# Autodesk Inventor assembly: assy-scara_new_components
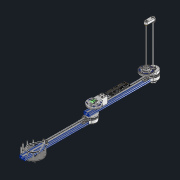
[picture p0: Inventor's stored thumbnail of the model, 180x180]
Saved by Autodesk Inventor 2022 (Build 260153000, 153)
## iProperties
Created: 2021-10-09
Part Number: assy-scara_new_components
Document SubType Name: Assembly
Designer: Yuta Kage
Mass: 10035.1 g
Surface Area: 20178.9 cm^2
Volume: 3427.41 cm^3
Density: 2.92791 g/cm^3
Author: Yuta Kage
## Documents named in this file (5)
- C:\Users\yuta0\Desktop\assy-scara\assy-scara_new_components.iam
- C:\Users\yuta0\Desktop\assy-scara\s-assy-linear_joint.iam
- C:\Users\yuta0\Desktop\assy-scara\s-assy-scara_link2.iam
- C:\Users\yuta0\Desktop\assy-scara\s-assy-scara-link4.iam
- C:\Users\yuta0\Desktop\assy-scara\s-assy-scara_link1_components.iam
## Components (4 placed, 4 different names)
1. s-assy-scara_link1_components:1 [sub-assembly] — 角度:1, 角度:2, メイト:38, メイト:39
2. s-assy-scara_link2:1 [sub-assembly] — 角度:2, 角度:3, メイト:38, メイト:39, メイト:40, メイト:41
3. s-assy-linear_joint:1 [sub-assembly] — 角度:3, メイト:33, メイト:34, フラッシュ:1, メイト:40, メイト:41
4. s-assy-scara-link4:1 [sub-assembly] — メイト:33, メイト:34, フラッシュ:1
## Relationships (10: Mate 6, Angle 3, Flush 1)
- 角度:1 [Angle] (0 deg): s-assy-scara_link1_components:1
- 角度:2 [Angle] (180 deg): s-assy-scara_link1_components:1 ↔ s-assy-scara_link2:1
- 角度:3 [Angle] (180 deg): s-assy-scara_link2:1 ↔ s-assy-linear_joint:1
- フラッシュ:1 [Flush]: s-assy-linear_joint:1 ↔ s-assy-scara-link4:1
- メイト:33 [Mate]: s-assy-linear_joint:1 ↔ s-assy-scara-link4:1
- メイト:34 [Mate]: s-assy-linear_joint:1 ↔ s-assy-scara-link4:1
- メイト:38 [Mate]: s-assy-scara_link1_components:1 ↔ s-assy-scara_link2:1
- メイト:39 [Mate]: s-assy-scara_link1_components:1 ↔ s-assy-scara_link2:1
- メイト:40 [Mate]: s-assy-scara_link2:1 ↔ s-assy-linear_joint:1
- メイト:41 [Mate]: s-assy-scara_link2:1 ↔ s-assy-linear_joint:1
